# Autodesk Inventor assembly: wheel bearing 1764
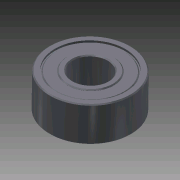
[picture p0: Inventor's stored thumbnail of the model, 180x180]
Saved by Autodesk Inventor 2011 (Build 150239000, 239)
## iProperties
Created: 2009-01-08
Part Number: wheel bearing 1764
Document SubType Name: Assembly
Designer: pmulligan
Author: pmulligan
## Documents named in this file (3)
- R:\CAD Archives\Wheels\Wheel bearing\wheel bearing 1764.iam
- R:\CAD Archives\Wheels\Wheel bearing\out casing 1764.ipt
- R:\CAD Archives\Wheels\Wheel bearing\inner ring 1764.ipt
## Components (2 placed, 2 different names)
1. out casing 1764:1 — Mate:1, Mate:2
2. inner ring 1764:1 — Mate:1, Mate:2, Angle:1, Mate:4
## Relationships (4: Mate 3, Angle 1)
- Mate:1: out casing 1764:1 ↔ inner ring 1764:1
- Mate:2: out casing 1764:1 ↔ inner ring 1764:1
- Angle:1 (0 deg): inner ring 1764:1
- Mate:4: inner ring 1764:1
